# Autodesk Inventor assembly: flute
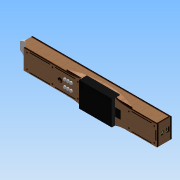
[picture p0: Inventor's stored thumbnail of the model, 180x180]
Saved by Autodesk Inventor 2015 (Build 190159000, 159)
## iProperties
Created: 2015-12-28
Part Number: flute
Document SubType Name: Assembly
Designer: Gregwar
Author: Gregwar
## Documents named in this file (11)
- C:\Users\Gregwar\Desktop\eFlute\3d\v1.1\flute.iam
- C:\Users\Gregwar\Desktop\eFlute\3d\v1.1\electronics.ipt
- C:\Users\Gregwar\Desktop\eFlute\3d\v1.1\bec.ipt
- C:\Users\Gregwar\Desktop\eFlute\3d\v1.1\top.ipt
- C:\Users\Gregwar\Desktop\eFlute\3d\v1.1\side.ipt
- C:\Users\Gregwar\Desktop\eFlute\3d\v1.1\bottom.ipt
- C:\Users\Gregwar\Desktop\eFlute\3d\v1.1\connectors.ipt
- C:\Users\Gregwar\Desktop\eFlute\3d\v1.1\bottom2.ipt
- C:\Users\Gregwar\Desktop\eFlute\3d\v1.1\button.ipt
- C:\Users\Gregwar\Desktop\eFlute\3d\v1.1\coffre.ipt
- C:\Users\Gregwar\Desktop\eFlute\3d\v1.1\side_sym.ipt
## Components (16 placed, 10 different names)
1. electronics:1 — Placage:1, Placage:2, Placage:3, Placage:19, Placage:20, Placage:21, Placage:22, Placage:23, Placage:24, Placage:25, Placage:26, Placage:27, Placage:28, Placage:29, Placage:30, Placage:38, Placage:42, Placage:43, Placage:45, Placage:46, Placage:48, Placage:49, Placage:51, Placage:52
2. bec:1 — Placage:1, Placage:2, Placage:3, Placage:4, Placage:5, Placage:6, Placage:10, Placage:11, Placage:36
3. top:1 — Placage:4, Placage:5, Placage:6, Placage:7, Affleurement:1, Affleurement:2, Placage:36, Placage:38, Placage:53, Placage:54, Placage:55, Placage:56, Placage:57, Affleurement:14, Affleurement:15, Placage:60
4. side:1 — Placage:7, Affleurement:1, Affleurement:2, Placage:41, Placage:47, Placage:53, Placage:54, Placage:55, Placage:63
5. bottom:1 — Placage:10, Placage:11, Placage:63
6. bottom2:1 — Placage:61, Affleurement:16, Placage:62
7. button:1 — Placage:19, Placage:20
8. button:2 — Placage:21, Placage:22
9. button:3 — Placage:23, Placage:24
10. button:4 — Placage:25, Placage:26
11. button:5 — Placage:27, Placage:28
12. button:6 — Placage:29, Placage:30
13. coffre:1 — Placage:41, Placage:42, Placage:43, Placage:47, Placage:48, Placage:49
14. coffre:2 — Placage:45, Placage:46, Placage:51, Placage:52, Placage:58
15. side_sym:1 — Placage:56, Placage:57, Affleurement:14, Placage:58, Placage:59, Placage:61
16. connectors:1 — Affleurement:15, Placage:59, Placage:60, Affleurement:16, Placage:62
## Relationships (49: Mate 44, Flush 5)
- Placage:1 [Mate]: electronics:1 ↔ bec:1
- Placage:2 [Mate]: electronics:1 ↔ bec:1
- Placage:3 [Mate]: electronics:1 ↔ bec:1
- Placage:4 [Mate]: bec:1 ↔ top:1
- Placage:5 [Mate]: bec:1 ↔ top:1
- Placage:6 [Mate]: bec:1 ↔ top:1
- Placage:7 [Mate]: top:1 ↔ side:1
- Affleurement:1 [Flush]: top:1 ↔ side:1
- Affleurement:2 [Flush]: top:1 ↔ side:1
- Placage:10 [Mate]: bec:1 ↔ bottom:1
- Placage:11 [Mate]: bec:1 ↔ bottom:1
- Placage:19 [Mate]: electronics:1 ↔ button:1
- Placage:20 [Mate]: electronics:1 ↔ button:1
- Placage:21 [Mate]: electronics:1 ↔ button:2
- Placage:22 [Mate]: electronics:1 ↔ button:2
- Placage:23 [Mate]: electronics:1 ↔ button:3
- Placage:24 [Mate]: electronics:1 ↔ button:3
- Placage:25 [Mate]: electronics:1 ↔ button:4
- Placage:26 [Mate]: electronics:1 ↔ button:4
- Placage:27 [Mate]: electronics:1 ↔ button:5
- Placage:28 [Mate]: electronics:1 ↔ button:5
- Placage:29 [Mate]: electronics:1 ↔ button:6
- Placage:30 [Mate]: electronics:1 ↔ button:6
- Placage:36 [Mate]: bec:1 ↔ top:1
- Placage:38 [Mate] (0.5 mm): electronics:1 ↔ top:1
- Placage:41 [Mate]: side:1 ↔ coffre:1
- Placage:42 [Mate]: electronics:1 ↔ coffre:1
- Placage:43 [Mate]: electronics:1 ↔ coffre:1
- Placage:45 [Mate]: electronics:1 ↔ coffre:2
- Placage:46 [Mate]: electronics:1 ↔ coffre:2
- Placage:47 [Mate]: side:1 ↔ coffre:1
- Placage:48 [Mate]: electronics:1 ↔ coffre:1
- Placage:49 [Mate]: electronics:1 ↔ coffre:1
- Placage:51 [Mate]: electronics:1 ↔ coffre:2
- Placage:52 [Mate]: electronics:1 ↔ coffre:2
- Placage:53 [Mate]: top:1 ↔ side:1
- Placage:54 [Mate]: top:1 ↔ side:1
- Placage:55 [Mate]: top:1 ↔ side:1
- Placage:56 [Mate]: top:1 ↔ side_sym:1
- Placage:57 [Mate]: top:1 ↔ side_sym:1
- Affleurement:14 [Flush]: top:1 ↔ side_sym:1
- Placage:58 [Mate]: coffre:2 ↔ side_sym:1
- Affleurement:15 [Flush]: top:1 ↔ connectors:1
- Placage:59 [Mate]: side_sym:1 ↔ connectors:1
- Placage:60 [Mate]: top:1 ↔ connectors:1
- Placage:61 [Mate]: bottom2:1 ↔ side_sym:1
- Affleurement:16 [Flush]: bottom2:1 ↔ connectors:1
- Placage:62 [Mate]: bottom2:1 ↔ connectors:1
- Placage:63 [Mate]: side:1 ↔ bottom:1
